# Autodesk Inventor assembly: XEndLeft
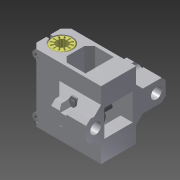
[picture p0: Inventor's stored thumbnail of the model, 180x180]
Saved by Autodesk Inventor 2015 (Build 190159000, 159)
## iProperties
Created: 2014-08-10
Part Number: XEndLeft
Document SubType Name: Assembly
Designer: Jack
Author: Jack
## Documents named in this file (9)
- C:\Users\t_clevj\ownCloud\CoreXY\InventorModel\XAxis\XEndVertLeft.iam
- C:\Users\t_clevj\ownCloud\CoreXY\InventorModel\XAxis\XEndVertRight.ipt
- C:\Users\t_clevj\ownCloud\CoreXY\InventorModel\Hardware\Bolts\SHCS\SHCS4\SHCS4x30.ipt
- C:\Users\t_clevj\ownCloud\CoreXY\InventorModel\Hardware\Nuts\Nut4.ipt
- C:\Users\t_clevj\ownCloud\CoreXY\InventorModel\Hardware\Bearing\Igus\BushingIgusRJM-01-08.ipt
- C:\Users\t_clevj\ownCloud\CoreXY\InventorModel\Hardware\Bolts\SHCS\SHCS3\SHCS3x25.ipt
- C:\Users\t_clevj\ownCloud\CoreXY\InventorModel\Hardware\Nuts\Nut3.ipt
- C:\Users\t_clevj\ownCloud\CoreXY\InventorModel\Hardware\Bearing\BearingRadialBall\BearingRadialBallF624zz.ipt
- C:\Users\t_clevj\ownCloud\CoreXY\InventorModel\Hardware\Wahsers\M4Washer.ipt
## Components (19 placed, 8 different names)
1. XEndVertRight:1 — Mate:6, Mate:7, Mate:8, Mate:9, Mate:11, Angle:1, Mate:13, Angle:2, Mate:25, Flush:1, Mate:26, Mate:39, Mate:40, Mate:44, Mate:45, Mate:47, Mate:48, Mate:49, Mate:50, Angle:3, Angle:4, Mate:64, Mate:66
2. SHCS4x30:1 — Mate:6, Mate:8, Mate:10, Mate:63
3. SHCS4x30:2 — Mate:7, Mate:9, Mate:12, Mate:65
4. Nut4:1 — Mate:10, Mate:11, Angle:1
5. Nut4:2 — Mate:12, Mate:13, Angle:2
6. BushingIgusRJM-01-08:1 — Mate:39, Mate:67
7. BushingIgusRJM-01-08:2 — Mate:40, Mate:68
8. SHCS3x25:1 — Mate:44, Mate:45, Mate:67
9. Nut3:1 — Mate:50, Angle:3
10. SHCS3x25:2 — Mate:47, Mate:48, Mate:68
11. Nut3:2 — Mate:49, Angle:4
12. BearingRadialBallF624zz:1
13. BearingRadialBallF624zz:2
14. M4Washer:1
15. M4Washer:2 — Mate:63, Mate:64
16. BearingRadialBallF624zz:3
17. BearingRadialBallF624zz:4
18. M4Washer:3
19. M4Washer:4 — Mate:65, Mate:66
## Relationships (43: Mate 38, Angle 4, Flush 1)
- Mate:6: XEndVertRight:1 ↔ SHCS4x30:1
- Mate:7: XEndVertRight:1 ↔ SHCS4x30:2
- Mate:8: XEndVertRight:1 ↔ SHCS4x30:1
- Mate:9: XEndVertRight:1 ↔ SHCS4x30:2
- Mate:10: SHCS4x30:1 ↔ Nut4:1
- Mate:11: XEndVertRight:1 ↔ Nut4:1
- Angle:1 (0 deg): XEndVertRight:1 ↔ Nut4:1
- Mate:12: SHCS4x30:2 ↔ Nut4:2
- Mate:13: XEndVertRight:1 ↔ Nut4:2
- Angle:2 (0 deg): XEndVertRight:1 ↔ Nut4:2
- Mate:25: XEndVertRight:1
- Flush:1: XEndVertRight:1
- Mate:26: XEndVertRight:1
- Mate:39: XEndVertRight:1 ↔ BushingIgusRJM-01-08:1
- Mate:40: XEndVertRight:1 ↔ BushingIgusRJM-01-08:2
- [Mate]: SHCS3x25:1 ↔ Nut3:1
- Mate:44: XEndVertRight:1 ↔ SHCS3x25:1
- Mate:45: XEndVertRight:1 ↔ SHCS3x25:1
- [Mate]: SHCS3x25:2 ↔ Nut3:2
- Mate:47: XEndVertRight:1 ↔ SHCS3x25:2
- Mate:48: XEndVertRight:1 ↔ SHCS3x25:2
- Mate:49: XEndVertRight:1 ↔ Nut3:2
- Mate:50: XEndVertRight:1 ↔ Nut3:1
- Angle:3 (0 deg): XEndVertRight:1 ↔ Nut3:1
- Angle:4 (0 deg): XEndVertRight:1 ↔ Nut3:2
- [Mate]: BearingRadialBallF624zz:1 ↔ BearingRadialBallF624zz:2
- [Mate]: BearingRadialBallF624zz:1 ↔ BearingRadialBallF624zz:2
- [Mate]: BearingRadialBallF624zz:1 ↔ M4Washer:1
- [Mate]: BearingRadialBallF624zz:2 ↔ M4Washer:1
- [Mate]: BearingRadialBallF624zz:1 ↔ M4Washer:2
- [Mate]: BearingRadialBallF624zz:1 ↔ M4Washer:2
- [Mate]: BearingRadialBallF624zz:3 ↔ BearingRadialBallF624zz:4
- [Mate]: BearingRadialBallF624zz:3 ↔ BearingRadialBallF624zz:4
- [Mate]: BearingRadialBallF624zz:3 ↔ M4Washer:3
- [Mate]: BearingRadialBallF624zz:4 ↔ M4Washer:3
- [Mate]: BearingRadialBallF624zz:3 ↔ M4Washer:4
- [Mate]: BearingRadialBallF624zz:3 ↔ M4Washer:4
- Mate:63: SHCS4x30:1 ↔ M4Washer:2
- Mate:64: XEndVertRight:1 ↔ M4Washer:2
- Mate:65: SHCS4x30:2 ↔ M4Washer:4
- Mate:66: XEndVertRight:1 ↔ M4Washer:4
- Mate:67: BushingIgusRJM-01-08:1 ↔ SHCS3x25:1
- Mate:68: BushingIgusRJM-01-08:2 ↔ SHCS3x25:2
## Named parameters: d51_d53 = 0 mm, d65_d160 = 0 mm, d66_d161 = 0 mm, d67_d162 = 0 mm, d68_d163 = 0 mm, d69_d158 = 0 mm, d70_d159 = 0 mm
